# Autodesk Inventor assembly: WHEEL ASSEMBLY
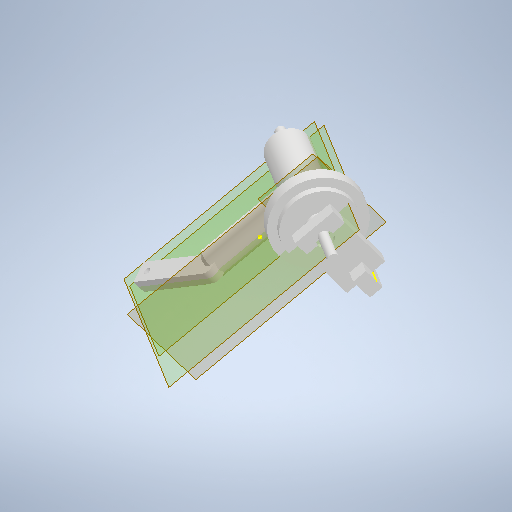
[picture p0: Inventor's stored thumbnail of the model, 512x512]
Saved by Autodesk Inventor 2025 (Build 290162010, 162A)
## iProperties
Created: 2024-08-26
Part Number: WHEEL ASSEMBLY
Document SubType Name: Assembly
Designer: darkb
Author: darkb
## Documents named in this file (4)
- C:\Users\darkb\Desktop\newpartsBRANDNEW\WHEEL ASSEMBLY.iam
- C:\Users\darkb\Desktop\newpartsBRANDNEW\NEWWHEELS.ipt
- C:\Users\darkb\Desktop\newpartsBRANDNEW\NEWYORKWHEELS.ipt
- C:\Users\darkb\Desktop\newpartsBRANDNEW\WHEEL RODS.ipt
## Components (3 placed, 3 different names)
1. NEWWHEELS:1 — Mate:1, Mate:2
2. NEWYORKWHEELS:1 — Mate:1
3. WHEEL RODS:1 — Mate:2
## Relationships (2: Mate 2)
- Mate:1: NEWWHEELS:1 ↔ NEWYORKWHEELS:1
- Mate:2: NEWWHEELS:1 ↔ WHEEL RODS:1
